# Autodesk Inventor assembly: 275-1272-001
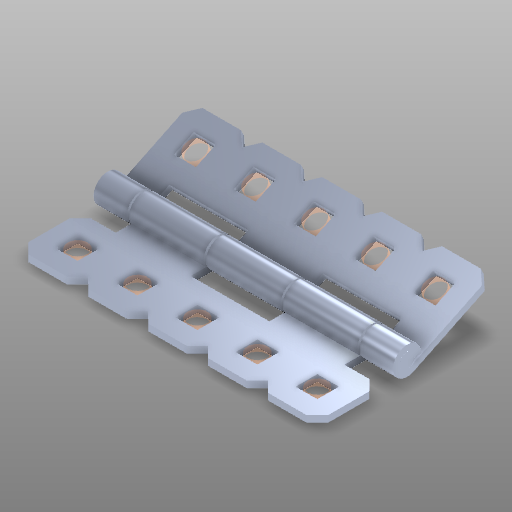
[picture p0: Inventor's stored thumbnail of the model, 512x512]
Saved by Autodesk Inventor 2021 (Build 250183000, 183)
## iProperties
Category: Structure
Company: Super Sonic Sparks, Team 24
Part Number: 275-1272-001
Document SubType Name: Assembly
Designer: Jordan Kiesel
Catalog Web Link: vexrobotics.com/275-1272.html
Description: Provides a simple pivoting joint.
Vendor: VEX Robotics, Inc.
Mass: 29.4658 g
Surface Area: 66.2962 cm^2
Volume: 4.04593 cm^3
Density: 7.28282 g/cm^3
Created: 2019-06-17
Translation Standard: STEP AP203
FileName: Hinge.iam
PreProcessor: SolidWorks 2010
PostProcessor: Build: 160, Release: 2012 RTM - Date: Tue 03/01/2011
Sent Units: inch
Uncertainty: 1e-05
Author: Jordan Kiesel
Title: Hinge
Comments: This hinge provides a simple pivoting joint with 265 degree movement. ▷ 2.5" long x 1.3" wide. ▷ Standard VEX holes.
## Documents named in this file (4)
- E:\VEX Cad\Library 1.1\Motion\Hinges\Hinge 5 Holes.iam
- E:\VEX Cad\Library 1.1\Motion\Hinges\Reference Parts\5 Holes\Pin 5.ipt
- E:\VEX Cad\Library 1.1\Motion\Hinges\Reference Parts\5 Holes\Bottom 5.ipt
- E:\VEX Cad\Library 1.1\Motion\Hinges\Reference Parts\5 Holes\Top 5.ipt
## Components (3 placed, 3 different names)
1. Bottom 5:1 — Mate:2, Mate:3
2. Pin 5:1 — Flush:1, Mate:1, Mate:3
3. Top 5:1 — Flush:1, Mate:1, Mate:2
## Relationships (4: Mate 3, Flush 1)
- Flush:1: Pin 5:1 ↔ Top 5:1
- Mate:1: Pin 5:1 ↔ Top 5:1
- Mate:2 (0.4064 mm): Bottom 5:1 ↔ Top 5:1
- Mate:3: Bottom 5:1 ↔ Pin 5:1
